# Autodesk Inventor assembly: back_holder
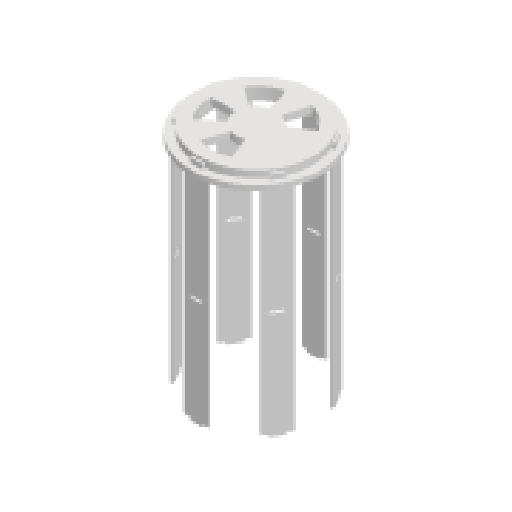
[picture p0: Inventor's stored thumbnail of the model, 512x512]
Saved by Autodesk Inventor 2024 (Build 280153000, 153)
## iProperties
Created: 2024-03-23
Part Number: back_holder
Document SubType Name: Assembly
Designer: op04o
Author: op04o
## Documents named in this file (4)
- C:\Users\op04o\OneDrive\桌面\實務\upper_holder\back_holder.iam
- C:\Users\op04o\OneDrive\桌面\實務\upper_holder\back_down_hold.ipt
- C:\Users\op04o\OneDrive\桌面\實務\upper_holder\back_cir_hold.ipt
- C:\Users\op04o\OneDrive\桌面\實務\upper_holder\back_cir_hold2.ipt
## Components (8 placed, 3 different names)
1. back_down_hold:1 — Mate:1, Mate:2, Mate:4
2. back_down_hold:2 — Mate:3, Mate:5, Mate:6
3. back_down_hold:3 — Mate:10, Mate:12, Mate:17
4. back_down_hold:4 — Mate:9, Mate:11, Mate:18
5. back_down_hold:5 — Mate:7, Mate:14, Mate:15
6. back_down_hold:6 — Mate:8, Mate:13, Mate:16
7. back_cir_hold:1 — Mate:1, Mate:2, Mate:3, Mate:4, Mate:5, Mate:6, Mate:7, Mate:8, Mate:9, Mate:10, Mate:11, Mate:12, Mate:13, Mate:14, Mate:15, Mate:16, Mate:17, Mate:18, Mate:19, Mate:20
8. back_cir_hold2:1 — Mate:19, Mate:20
## Relationships (20: Mate 20)
- Mate:1: back_down_hold:1 ↔ back_cir_hold:1
- Mate:2: back_down_hold:1 ↔ back_cir_hold:1
- Mate:3: back_down_hold:2 ↔ back_cir_hold:1
- Mate:4: back_down_hold:1 ↔ back_cir_hold:1
- Mate:5: back_down_hold:2 ↔ back_cir_hold:1
- Mate:6: back_down_hold:2 ↔ back_cir_hold:1
- Mate:7: back_down_hold:5 ↔ back_cir_hold:1
- Mate:8: back_down_hold:6 ↔ back_cir_hold:1
- Mate:9: back_down_hold:4 ↔ back_cir_hold:1
- Mate:10: back_down_hold:3 ↔ back_cir_hold:1
- Mate:11: back_down_hold:4 ↔ back_cir_hold:1
- Mate:12: back_down_hold:3 ↔ back_cir_hold:1
- Mate:13: back_down_hold:6 ↔ back_cir_hold:1
- Mate:14: back_down_hold:5 ↔ back_cir_hold:1
- Mate:15: back_down_hold:5 ↔ back_cir_hold:1
- Mate:16: back_down_hold:6 ↔ back_cir_hold:1
- Mate:17: back_down_hold:3 ↔ back_cir_hold:1
- Mate:18: back_down_hold:4 ↔ back_cir_hold:1
- Mate:19: back_cir_hold:1 ↔ back_cir_hold2:1
- Mate:20: back_cir_hold:1 ↔ back_cir_hold2:1
